# Autodesk Inventor assembly: Universal Shaft
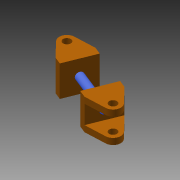
[picture p0: Inventor's stored thumbnail of the model, 180x180]
Saved by Autodesk Inventor 2016 (Build 200138000, 138)
## iProperties
Created: 2014-03-11
Part Number: Universal Shaft
Document SubType Name: Assembly
Designer: John
Author: John
## Documents named in this file (3)
- C:\File Storage\Autodesk\Inventor 2016 Projects\Ex_Files_Inventor_2016_EssT\Exercise Files\15_Using constraints to position parts\15_01\Universal Shaft.iam
- C:\File Storage\Autodesk\Inventor 2016 Projects\Ex_Files_Inventor_2016_EssT\Exercise Files\14_Adding parts to an assembly file\14_01\Joint.ipt
- C:\File Storage\Autodesk\Inventor 2016 Projects\Ex_Files_Inventor_2016_EssT\Exercise Files\14_Adding parts to an assembly file\14_01\Connecting Rod.ipt
## Components (3 placed, 2 different names)
1. Joint:1 — Flush:3
2. Joint:2
3. Connecting Rod:1 — Flush:3
## Relationships (5: Flush 3, Mate 2)
- [Mate]: Joint:1 ↔ Joint:2
- [Flush]: Joint:1 ↔ Joint:2
- [Mate]: Joint:1 ↔ Connecting Rod:1
- [Flush]: Joint:2 ↔ Connecting Rod:1
- Flush:3: Joint:1 ↔ Connecting Rod:1
